# Autodesk Inventor assembly: Switch_Micro-L
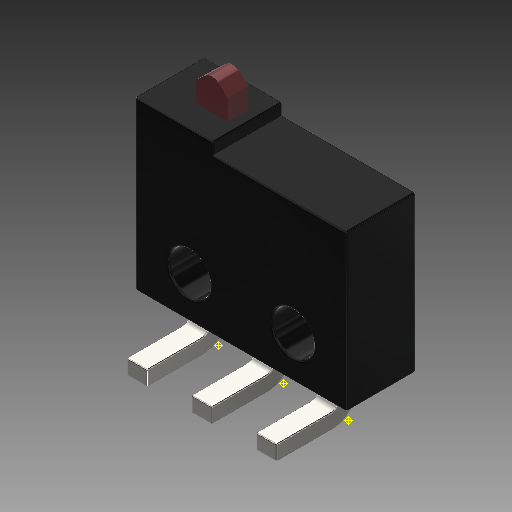
[picture p0: Inventor's stored thumbnail of the model, 512x512]
Saved by Autodesk Inventor 2018 (Build 220112000, 112)
## iProperties
Created: 2013-07-18
Part Number: Switch_Micro-L
Document SubType Name: Assembly
Designer: Bradley
Sending System: SolidWorks 2002025
Preprocessor: SwSTEP 2.0
## Documents named in this file (3)
- C:\Users\Bradley\Documents\GitHub\Resources\SupplierDocuments\49 - Electromechanical\49-0001\49-0001.iam
- C:\Users\Bradley\Documents\GitHub\Resources\SupplierDocuments\49 - Electromechanical\49-0001\D2MQ_1_TL_ACTUATOR.ipt
- C:\Users\Bradley\Documents\GitHub\Resources\SupplierDocuments\49 - Electromechanical\49-0001\D2MQ_1_TL_BASE.ipt
## Components (2 placed, 2 different names)
1. D2MQ_1_TL_ACTUATOR_1 — Flush:1, Flush:2, Mate:1
2. D2MQ_1_TL_BASE_2 — Flush:1, Flush:2, Mate:1, Flush:3, Flush:4, Mate:2
## Relationships (6: Flush 4, Mate 2)
- Flush:1 (-0.95 mm): D2MQ_1_TL_ACTUATOR_1 ↔ D2MQ_1_TL_BASE_2
- Flush:2 (-1.45 mm): D2MQ_1_TL_ACTUATOR_1 ↔ D2MQ_1_TL_BASE_2
- Mate:1 (-6.1 mm): D2MQ_1_TL_ACTUATOR_1 ↔ D2MQ_1_TL_BASE_2
- Flush:3: D2MQ_1_TL_BASE_2
- Flush:4: D2MQ_1_TL_BASE_2
- Mate:2 (-4.1 mm): D2MQ_1_TL_BASE_2
